# Autodesk Inventor assembly: !drivebay
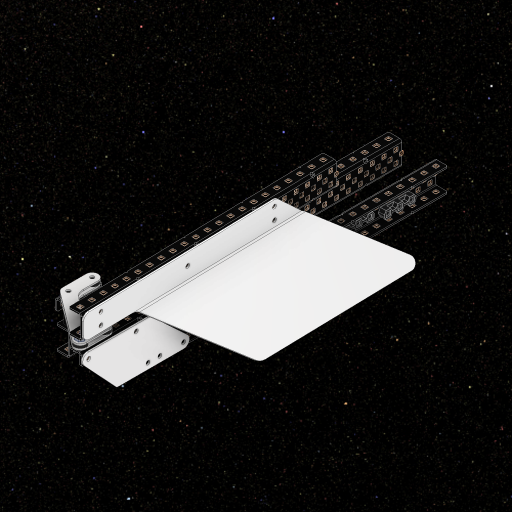
[picture p0: Inventor's stored thumbnail of the model, 512x512]
Saved by Autodesk Inventor 2024 (Build 280153000, 153)
## iProperties
Created: 2024-02-24
Part Number: !drivebay
Document SubType Name: Assembly
Designer: Averey Ku
Author: Averey Ku
## Documents named in this file (13)
- D:\vex_robotics\hardware\cad\lil_zoom\custom_parts\chassis\drivebay\!drivebay.iam
- D:\vex_robotics\hardware\cad\lil_zoom\chassis\drivebay\outer.iam
- D:\vex_robotics\hardware\cad\lil_zoom\chassis\drivebay\inner.iam
- D:\vex_robotics\hardware\cad\lil_zoom\custom_parts\chassis\drivebay\gusset.ipt
- D:\vex_robotics\hardware\cad\VEX-CAD-Inventor-1.41\Motion\Spacers\Spacer Nylon .500 OD\NSpacer Black .500 OD x .125.ipt
- D:\vex_robotics\hardware\cad\VEX-CAD-Inventor-1.41\Motion\Spacers\Spacer Nylon .500 OD.ipt
- D:\vex_robotics\hardware\cad\VEX-CAD-Inventor-1.41\Structure\Standoff\Standoff 2.50.ipt
- D:\vex_robotics\hardware\cad\VEX-CAD-Inventor-1.41\Structure\Standoff.ipt
- D:\vex_robotics\hardware\cad\VEX-CAD-Inventor-1.41\Structure\Hardware\Nut Thin Nylock.ipt
- D:\vex_robotics\hardware\cad\VEX-CAD-Inventor-1.41\Structure\C Channel\Aluminum 1x2x1\Alu C 1x2x1x22.ipt
- D:\vex_robotics\hardware\cad\lil_zoom\custom_parts\chassis\drivebay\wing.ipt
- D:\vex_robotics\hardware\cad\VEX-CAD-Inventor-1.41\Structure\Standoff\Standoff 1.25.ipt
- D:\vex_robotics\hardware\cad\VEX-CAD-Inventor-1.41\Motion\Spacers\Washer Delrin\DWasher .500 OD x .062500.ipt
## Components (15 placed, 10 different names)
1. outer:1 [sub-assembly] — Insert:1, Mate:1, Insert:2, Mate:2, Insert:14, Mate:6
2. inner:1 [sub-assembly] — Insert:1, Mate:1, Mate:4, Insert:20
3. gusset:1 — Insert:2, Mate:2, Insert:3, Mate:3
4. gusset:2 — Insert:3, Mate:3, Insert:4, Insert:5, Insert:6, Insert:7, Insert:15
5. NSpacer Black .500 OD x .125:1 — Insert:5
6. NSpacer Black .500 OD x .125:2 — Insert:4
7. NSpacer Black .500 OD x .125:3 — Insert:6
8. NSpacer Black .500 OD x .125:4 — Insert:7
9. Standoff 2.50:1 — Insert:14, Mate:4
10. Nut Thin Nylock:1 — Insert:15, Insert:16
11. Alu C 1x2x1x22:1 — Insert:16, Insert:17, Mate:5
12. wing:1 — Insert:17, Mate:5
13. Standoff 1.25:1 — Insert:18, Insert:19
14. DWasher .500 OD x .062500:1 — Insert:19, Insert:20
15. DWasher .500 OD x .062500:2 — Insert:18, Mate:6
## Relationships (20: Insert 14, Mate 6)
- Insert:1 (34.925 mm): outer:1 ↔ inner:1
- Mate:1: outer:1 ↔ inner:1
- Insert:2: outer:1 ↔ gusset:1
- Mate:2: outer:1 ↔ gusset:1
- Insert:3 (3.175 mm): gusset:1 ↔ gusset:2
- Mate:3: gusset:1 ↔ gusset:2
- Insert:4: gusset:2 ↔ NSpacer Black .500 OD x .125:2
- Insert:5: gusset:2 ↔ NSpacer Black .500 OD x .125:1
- Insert:6: gusset:2 ↔ NSpacer Black .500 OD x .125:3
- Insert:7: gusset:2 ↔ NSpacer Black .500 OD x .125:4
- Insert:14: outer:1 ↔ Standoff 2.50:1
- Mate:4: inner:1 ↔ Standoff 2.50:1
- Insert:15: gusset:2 ↔ Nut Thin Nylock:1
- Insert:16: Nut Thin Nylock:1 ↔ Alu C 1x2x1x22:1
- Insert:17: Alu C 1x2x1x22:1 ↔ wing:1
- Mate:5: Alu C 1x2x1x22:1 ↔ wing:1
- Insert:18: Standoff 1.25:1 ↔ DWasher .500 OD x .062500:2
- Insert:19: Standoff 1.25:1 ↔ DWasher .500 OD x .062500:1
- Insert:20: inner:1 ↔ DWasher .500 OD x .062500:1
- Mate:6: outer:1 ↔ DWasher .500 OD x .062500:2
